# Autodesk Inventor assembly: Rocker
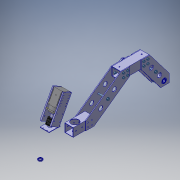
[picture p0: Inventor's stored thumbnail of the model, 180x180]
Saved by Autodesk Inventor 2018 (Build 220112000, 112)
## iProperties
Created: 2017-09-12
Part Number: Rocker
Material: 一般
Document SubType Name: Assembly
Designer: 翔
Source: UnKnown
Author: 翔
## Documents named in this file (19)
- E:\forest_robot_cad\fr03\Rocker.iam
- E:\forest_robot_cad\terzo tentativo\flange_rocker.ipt
- E:\forest_robot_cad\terzo tentativo\rocker_up.ipt
- E:\forest_robot_cad\terzo tentativo\B6802ZZ_2_03.ipt
- E:\forest_robot_cad\terzo tentativo\bogie_flange_to_rocker.ipt
- E:\forest_robot_cad\terzo tentativo\bogie_flange_to_rocker_2.ipt
- E:\forest_robot_cad\terzo tentativo\holder_rocker_shaft.ipt
- E:\forest_robot_cad\terzo tentativo\Revolute_joint_bearing_holder.ipt
- E:\forest_robot_cad\terzo tentativo\boltM6_rockerflange.iam
- E:\forest_robot_cad\terzo tentativo\BoltM6flangerevolutejoint.iam
- E:\forest_robot_cad\terzo tentativo\Reinforce_rocker_up.ipt
- E:\forest_robot_cad\terzo tentativo\boltM8reinforcedpipe.iam
- E:\forest_robot_cad\terzo tentativo\L54-30-S400-R.ipt
- E:\forest_robot_cad\terzo tentativo\flange.ipt
- E:\forest_robot_cad\terzo tentativo\Product23.iam
- E:\forest_robot_cad\terzo tentativo\shaft support coupling.ipt
- E:\forest_robot_cad\terzo tentativo\support new servomotor.ipt
- E:\forest_robot_cad\terzo tentativo\help plate 2.ipt
- E:\forest_robot_cad\fr03\rocker_arm.ipt
## Components (48 placed, 47 different names)
1. flange_rocker.1 — メイト:12, フラッシュ:2, メイト:13, メイト:14
2. rocker_up.1 — メイト:12, フラッシュ:2, メイト:13
3. _B6802ZZ.1
4. bogie_flange_to_rocker.1
5. bogie_flange_to_rocker_2.1
6. holder_rocker_shaft.1
7. revolute_joint_bearing.1
8. _B6802ZZ.3
9. _B6802ZZ.4
10. _B6802ZZ.5
11. _B6802ZZ.6
12. boltM6_rockerflange.1 [sub-assembly]
13. boltM6_rockerflange.2 [sub-assembly]
14. boltM6_rockerflange.3 [sub-assembly]
15. boltM6_rockerflange.4 [sub-assembly]
16. boltM6_rockerflange.5 [sub-assembly]
17. boltM6_rockerflange.6 [sub-assembly]
18. boltM6_rockerflange.7 [sub-assembly]
19. boltM6_rockerflange.8 [sub-assembly]
20. boltM6_rockerflange.12 [sub-assembly]
21. boltM6_rockerflange.14 [sub-assembly]
22. boltM6_rockerflange.15 [sub-assembly]
23. boltM6_rockerflange.16 [sub-assembly]
24. BoltM6flangerevolutejoint.1 [sub-assembly]
25. BoltM6flangerevolutejoint.2 [sub-assembly]
26. BoltM6flangerevolutejoint.3 [sub-assembly]
27. BoltM6flangerevolutejoint.4 [sub-assembly]
28. Reinforce_rocker_up.1
29. Reinforce_rocker_up.2
30. flange_rocker.2 — フラッシュ:3, メイト:15
31. boltM6_rockerflange.9 [sub-assembly]
32. boltM6_rockerflange.10 [sub-assembly]
33. boltM6_rockerflange.11 [sub-assembly]
34. boltM6_rockerflange.17 [sub-assembly]
35. boltM6_rockerflange.18 [sub-assembly]
36. boltM6_rockerflange.19 [sub-assembly]
37. boltM6_rockerflange.20 [sub-assembly]
38. boltM6_rockerflange.21 [sub-assembly]
39. boltM8reinforcedpipe.1 [sub-assembly]
40. boltM8reinforcedpipe.2 [sub-assembly]
41. L54-30-S400-R:1 — メイト:1, メイト:2, メイト:3, メイト:6, メイト:7, メイト:8, メイト:9, メイト:10, メイト:11
42. flange:1 — メイト:1, メイト:2, メイト:3, メイト:4
43. Product23:1 [sub-assembly] — メイト:4, メイト:5
44. shaft support coupling:1 — メイト:5
45. support new servomotor:1 — メイト:6, メイト:7, メイト:8
46. help plate 2:1
47. support new servomotor:2 — メイト:9, メイト:10, メイト:11
48. rocker_arm:1 — メイト:14, フラッシュ:3, メイト:15
## Relationships (17: Mate 15, Flush 2)
- メイト:1 [Mate]: L54-30-S400-R:1 ↔ flange:1
- メイト:2 [Mate]: L54-30-S400-R:1 ↔ flange:1
- メイト:3 [Mate]: L54-30-S400-R:1 ↔ flange:1
- メイト:4 [Mate]: flange:1 ↔ Product23:1
- メイト:5 [Mate]: Product23:1 ↔ shaft support coupling:1
- メイト:6 [Mate]: L54-30-S400-R:1 ↔ support new servomotor:1
- メイト:7 [Mate]: L54-30-S400-R:1 ↔ support new servomotor:1
- メイト:8 [Mate]: L54-30-S400-R:1 ↔ support new servomotor:1
- メイト:9 [Mate]: L54-30-S400-R:1 ↔ support new servomotor:2
- メイト:10 [Mate]: L54-30-S400-R:1 ↔ support new servomotor:2
- メイト:11 [Mate]: L54-30-S400-R:1 ↔ support new servomotor:2
- メイト:12 [Mate]: flange_rocker.1 ↔ rocker_up.1
- フラッシュ:2 [Flush]: flange_rocker.1 ↔ rocker_up.1
- メイト:13 [Mate]: flange_rocker.1 ↔ rocker_up.1
- メイト:14 [Mate]: flange_rocker.1 ↔ rocker_arm:1
- フラッシュ:3 [Flush]: flange_rocker.2 ↔ rocker_arm:1
- メイト:15 [Mate]: flange_rocker.2 ↔ rocker_arm:1
